# Autodesk Inventor assembly: floor
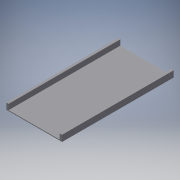
[picture p0: Inventor's stored thumbnail of the model, 180x180]
Saved by Autodesk Inventor 2017 (Build 210142000, 142)
## iProperties
Created: 2019-05-05
Part Number: floor
Document SubType Name: Assembly
Designer: Roman
Author: Roman
## Documents named in this file (3)
- C:\Users\Roman\Documents\CAD\tegu rev2\floor\floor.iam
- C:\Users\Roman\Documents\CAD\tegu rev2\floor\floor back.ipt
- C:\Users\Roman\Documents\CAD\tegu rev2\floor\floor long 2x4.ipt
## Components (3 placed, 2 different names)
1. floor back:1 — Mate:1, Mate:2, Flush:1, Flush:2, Flush:3, Flush:4
2. floor long 2x4:1 — Mate:2, Flush:1, Flush:3
3. floor long 2x4:2 — Mate:1, Flush:2, Flush:4
## Relationships (6: Flush 4, Mate 2)
- Mate:1: floor back:1 ↔ floor long 2x4:2
- Mate:2: floor back:1 ↔ floor long 2x4:1
- Flush:1: floor back:1 ↔ floor long 2x4:1
- Flush:2: floor back:1 ↔ floor long 2x4:2
- Flush:3: floor back:1 ↔ floor long 2x4:1
- Flush:4: floor back:1 ↔ floor long 2x4:2
